# Autodesk Inventor assembly: Полигон
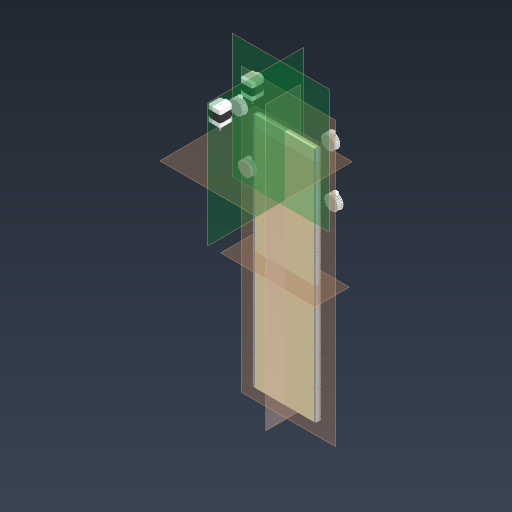
[picture p0: Inventor's stored thumbnail of the model, 512x512]
Saved by Autodesk Inventor 2023.2 (Build 272271030, 271C)
## iProperties
Created: 2025-12-08
Part Number: Полигон
Document SubType Name: Assembly
Designer: Олег Коноваленко
Author: Олег Коноваленко
## Documents named in this file (4)
- D:\VSOSH_IT_Robotics_ETZ\ETZ\Сonstruction\Полигон.iam
- D:\VSOSH_IT_Robotics_ETZ\ETZ\Сonstruction\Вертикальная_поверхность.ipt
- C:\Users\I9232\Downloads\m2_20\m2_20.ipt
- D:\VSOSH_IT_Robotics_ETZ\ETZ\Сonstruction\Робот_ЕТЗ.iam
## Components (10 placed, 3 different names)
1. Вертикальная_поверхность:1 — Совмещение:1, Совмещение:2, Совмещение:3, Совмещение:4, Совмещение:5, Совмещение:6, Совмещение:7, Совмещение:8, Заподлицо:1, Заподлицо:2, Заподлицо:3, Заподлицо:4, Заподлицо:5, Заподлицо:6, Заподлицо:7, Заподлицо:8, Заподлицо:9, Заподлицо:10, Совмещение:15, Совмещение:16, Заподлицо:11
2. Робот_ЕТЗ:1 [sub-assembly] — Совмещение:17
3. m2_20:1 — Совмещение:2, Заподлицо:9, Совмещение:12, Совмещение:13
4. m2_20:2 — Совмещение:1, Совмещение:13, Заподлицо:10
5. m2_20:3 — Совмещение:3, Совмещение:11, Заподлицо:8, Совмещение:12
6. m2_20:4 — Совмещение:4, Заподлицо:6, Совмещение:11, Заподлицо:7
7. m2_20:5 — Совмещение:5, Заподлицо:1, Совмещение:14
8. m2_20:6 — Совмещение:6, Заподлицо:2, Совмещение:10, Совмещение:14
9. m2_20:7 — Совмещение:7, Заподлицо:4, Совмещение:9, Совмещение:10
10. m2_20:8 — Совмещение:8, Заподлицо:3, Заподлицо:5, Совмещение:9
## Relationships (28: Mate 17, Flush 11)
- Совмещение:1 [Mate]: Вертикальная_поверхность:1 ↔ m2_20:2
- Совмещение:2 [Mate]: Вертикальная_поверхность:1 ↔ m2_20:1
- Совмещение:3 [Mate]: Вертикальная_поверхность:1 ↔ m2_20:3
- Совмещение:4 [Mate]: Вертикальная_поверхность:1 ↔ m2_20:4
- Совмещение:5 [Mate]: Вертикальная_поверхность:1 ↔ m2_20:5
- Совмещение:6 [Mate]: Вертикальная_поверхность:1 ↔ m2_20:6
- Совмещение:7 [Mate]: Вертикальная_поверхность:1 ↔ m2_20:7
- Совмещение:8 [Mate]: Вертикальная_поверхность:1 ↔ m2_20:8
- Заподлицо:1 [Flush]: Вертикальная_поверхность:1 ↔ m2_20:5
- Заподлицо:2 [Flush]: Вертикальная_поверхность:1 ↔ m2_20:6
- Заподлицо:3 [Flush]: Вертикальная_поверхность:1 ↔ m2_20:8
- Заподлицо:4 [Flush]: Вертикальная_поверхность:1 ↔ m2_20:7
- Заподлицо:5 [Flush]: Вертикальная_поверхность:1 ↔ m2_20:8
- Совмещение:9 [Mate]: m2_20:7 ↔ m2_20:8
- Совмещение:10 [Mate]: m2_20:6 ↔ m2_20:7
- Заподлицо:6 [Flush]: Вертикальная_поверхность:1 ↔ m2_20:4
- Совмещение:11 [Mate]: m2_20:3 ↔ m2_20:4
- Заподлицо:7 [Flush]: Вертикальная_поверхность:1 ↔ m2_20:4
- Заподлицо:8 [Flush]: Вертикальная_поверхность:1 ↔ m2_20:3
- Заподлицо:9 [Flush]: Вертикальная_поверхность:1 ↔ m2_20:1
- Совмещение:12 [Mate]: m2_20:1 ↔ m2_20:3
- Совмещение:13 [Mate]: m2_20:1 ↔ m2_20:2
- Заподлицо:10 [Flush]: Вертикальная_поверхность:1 ↔ m2_20:2
- Совмещение:14 [Mate]: m2_20:5 ↔ m2_20:6
- Совмещение:15 [Mate]: Вертикальная_поверхность:1
- Совмещение:16 [Mate]: Вертикальная_поверхность:1
- Заподлицо:11 [Flush]: Вертикальная_поверхность:1
- Совмещение:17 [Mate]: Робот_ЕТЗ:1
